# Autodesk Inventor assembly: Chuck Assembly
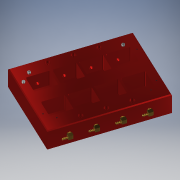
[picture p0: Inventor's stored thumbnail of the model, 180x180]
Saved by Autodesk Inventor 2019.4 (Build 234330000, 330)
## iProperties
Created: 2021-01-11
Part Number: Chuck Assembly
Document SubType Name: Assembly
Designer: caleb
Author: caleb
## Documents named in this file (4)
- C:\Users\cfang\Desktop\nebraska-silicon-lab\Hardware\ETL\Module Assembly\Chuck - Multipocket\Chuck Assembly.iam
- C:\Users\cfang\Desktop\nebraska-silicon-lab\Hardware\ETL\Module Assembly\Chuck - Multipocket\Chuck - Multipocket.ipt
- C:\Users\cfang\Desktop\nebraska-silicon-lab\Hardware\ETL\Module Assembly\Chuck - Multipocket\90128A212_ZNC-PLTD ALLOY STL SCKT HEAD CAP SCREW.ipt
- C:\Users\cfang\Desktop\nebraska-silicon-lab\Hardware\ETL\Module Assembly\Chuck - Multipocket\44555K147_BRASS BARBED TUBE FITTING FOR VACUUM.ipt
## Components (12 placed, 3 different names)
1. Chuck - Multipocket:1 — Insert:1, Insert:2, Insert:3, Insert:6, Insert:7, Insert:8, Insert:9, Insert:10, Insert:11, Insert:12, Insert:13
2. 90128A212_ZNC-PLTD ALLOY STL SCKT HEAD CAP SCREW:1 — Insert:2
3. 90128A212_ZNC-PLTD ALLOY STL SCKT HEAD CAP SCREW:2 — Insert:3
4. 90128A212_ZNC-PLTD ALLOY STL SCKT HEAD CAP SCREW:3 — Insert:1
5. 44555K147_BRASS BARBED TUBE FITTING FOR VACUUM:1 — Insert:7
6. 44555K147_BRASS BARBED TUBE FITTING FOR VACUUM:2 — Insert:10
7. 44555K147_BRASS BARBED TUBE FITTING FOR VACUUM:3 — Insert:11
8. 44555K147_BRASS BARBED TUBE FITTING FOR VACUUM:4 — Insert:12
9. 44555K147_BRASS BARBED TUBE FITTING FOR VACUUM:5 — Insert:13
10. 44555K147_BRASS BARBED TUBE FITTING FOR VACUUM:6 — Insert:9
11. 44555K147_BRASS BARBED TUBE FITTING FOR VACUUM:7 — Insert:8
12. 44555K147_BRASS BARBED TUBE FITTING FOR VACUUM:8 — Insert:6
## Relationships (11: Insert 11)
- Insert:1: Chuck - Multipocket:1 ↔ 90128A212_ZNC-PLTD ALLOY STL SCKT HEAD CAP SCREW:3
- Insert:2: Chuck - Multipocket:1 ↔ 90128A212_ZNC-PLTD ALLOY STL SCKT HEAD CAP SCREW:1
- Insert:3: Chuck - Multipocket:1 ↔ 90128A212_ZNC-PLTD ALLOY STL SCKT HEAD CAP SCREW:2
- Insert:6: Chuck - Multipocket:1 ↔ 44555K147_BRASS BARBED TUBE FITTING FOR VACUUM:8
- Insert:7: Chuck - Multipocket:1 ↔ 44555K147_BRASS BARBED TUBE FITTING FOR VACUUM:1
- Insert:8: Chuck - Multipocket:1 ↔ 44555K147_BRASS BARBED TUBE FITTING FOR VACUUM:7
- Insert:9: Chuck - Multipocket:1 ↔ 44555K147_BRASS BARBED TUBE FITTING FOR VACUUM:6
- Insert:10: Chuck - Multipocket:1 ↔ 44555K147_BRASS BARBED TUBE FITTING FOR VACUUM:2
- Insert:11: Chuck - Multipocket:1 ↔ 44555K147_BRASS BARBED TUBE FITTING FOR VACUUM:3
- Insert:12: Chuck - Multipocket:1 ↔ 44555K147_BRASS BARBED TUBE FITTING FOR VACUUM:4
- Insert:13: Chuck - Multipocket:1 ↔ 44555K147_BRASS BARBED TUBE FITTING FOR VACUUM:5
